# Autodesk Inventor assembly: Flyver
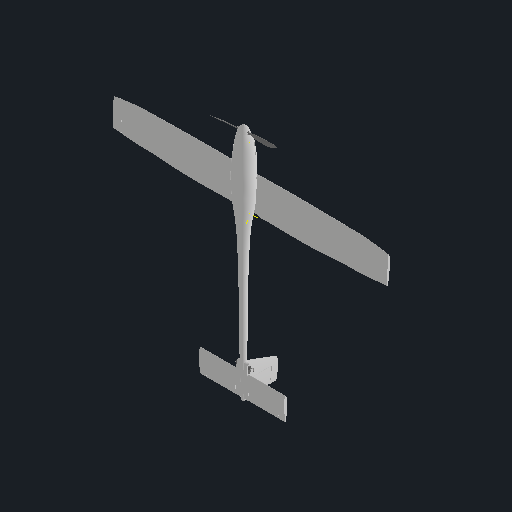
[picture p0: Inventor's stored thumbnail of the model, 512x512]
Saved by Autodesk Inventor 2026.2 (Build 302298000, 298)
## iProperties
Created: 2021-04-28
Part Number: Flyver
Document SubType Name: Assembly
Designer: armin
Author: armin
## Documents named in this file (19)
- C:\Users\Malthe Sennels\OneDrive - Aalborg Universitet\ESD 610 - General\Inventor\Cover_image\Flyver\Flyver.iam
- C:\Users\Malthe Sennels\OneDrive - Aalborg Universitet\ESD 610 - General\Inventor\Cover_image\Flyver\Body hollow.ipt
- C:\Users\Malthe Sennels\OneDrive - Aalborg Universitet\ESD 610 - General\Inventor\Cover_image\Flyver\Avionics.iam
- C:\Users\Malthe Sennels\OneDrive - Aalborg Universitet\ESD 610 - General\Inventor\Cover_image\Flyver\Wing.ipt
- C:\Users\Malthe Sennels\OneDrive - Aalborg Universitet\ESD 610 - General\Inventor\Cover_image\Flyver\Tunnel.ipt
- C:\Users\Malthe Sennels\OneDrive - Aalborg Universitet\ESD 610 - General\Inventor\Cover_image\Flyver\Servo.ipt
- C:\Users\Malthe Sennels\OneDrive - Aalborg Universitet\ESD 610 - General\Inventor\Cover_image\Flyver\Rudder.ipt
- C:\Users\Malthe Sennels\OneDrive - Aalborg Universitet\ESD 610 - General\Inventor\Cover_image\Flyver\Rudder_MIR.ipt
- C:\Users\Malthe Sennels\OneDrive - Aalborg Universitet\ESD 610 - General\Inventor\Cover_image\Flyver\Servo arm.ipt
- C:\Users\Malthe Sennels\OneDrive - Aalborg Universitet\ESD 610 - General\Inventor\Cover_image\Flyver\Styrepind.ipt
- C:\Users\Malthe Sennels\OneDrive - Aalborg Universitet\ESD 610 - General\Inventor\Cover_image\Flyver\BLDC.ipt
- C:\Users\Malthe Sennels\OneDrive - Aalborg Universitet\ESD 610 - General\Inventor\Cover_image\Flyver\Propeller.iam
- C:\Users\Malthe Sennels\OneDrive - Aalborg Universitet\ESD 610 - General\Inventor\Cover_image\Flyver\Servo_MIR.ipt
- C:\Users\Malthe Sennels\OneDrive - Aalborg Universitet\ESD 610 - General\Inventor\Cover_image\Flyver\Servo arm_MIR.ipt
- C:\Users\Malthe Sennels\OneDrive - Aalborg Universitet\ESD 610 - General\Inventor\Cover_image\Flyver\Styrepind_MIR.ipt
- C:\Users\Malthe Sennels\OneDrive - Aalborg Universitet\ESD 610 - General\Inventor\Cover_image\Flyver\Tail.ipt
- C:\Users\Malthe Sennels\OneDrive - Aalborg Universitet\ESD 610 - General\Inventor\Cover_image\Flyver\Aileron.ipt
- C:\Users\Malthe Sennels\OneDrive - Aalborg Universitet\ESD 610 - General\Inventor\Cover_image\Flyver\Wing_MIR1.ipt
- C:\Users\Malthe Sennels\OneDrive - Aalborg Universitet\ESD 610 - General\Inventor\Cover_image\Flyver\Aileron_MIR.ipt
## Components (19 placed, 18 different names)
1. Body hollow:1 — Mate:1, Mate:2, Mate:14, Mate:16, Mate:17, Mate:18, Mate:19, Mate:20, Flush:2, Flush:4, Flush:5, Mate:31, Mate:37, Mate:38, Flush:7, Mate:41, Mate:42, Mate:51
2. Avionics:1 [sub-assembly] — Mate:1, Mate:2, Mate:3, Mate:4, Flush:1, Mate:8, Mate:48, Mate:49, Mate:50, Mate:51
3. Wing:1 — Mate:3, Mate:4, Mate:8, Mate:44, Mate:45
4. Tunnel:1
5. Servo:1 — Mate:19, Mate:20, Flush:2, Mate:21, Mate:22
6. Rudder:1 — Mate:14, Mate:16, Mate:24
7. Rudder_MIR:1 — Mate:17, Mate:18, Mate:39
8. Servo arm:1 — Mate:21, Mate:22, Mate:23, Flush:3
9. Styrepind:1 — Mate:23, Mate:24, Flush:3
10. BLDC:1 — Mate:26, Mate:27, Mate:31, Mate:32, Mate:33, Mate:41
11. Propeller:1 [sub-assembly] — Mate:32, Mate:33
12. Servo_MIR:1 — Mate:34, Mate:35, Mate:37, Mate:38, Flush:7
13. Servo arm_MIR:1 — Mate:34, Mate:35, Flush:6, Mate:36
14. Styrepind_MIR:1 — Flush:6, Mate:36, Mate:39
15. Tail:1 — Mate:42
16. Aileron:1 — Mate:44, Mate:45
17. Wing_MIR1:1 — Mate:46, Mate:47, Mate:48, Mate:49, Mate:50
18. Aileron_MIR:1 — Mate:46, Mate:47
19. Tunnel:2
## Relationships (43: Mate 36, Flush 7)
- Mate:1: Body hollow:1 ↔ Avionics:1
- Mate:2: Body hollow:1 ↔ Avionics:1
- Mate:3: Avionics:1 ↔ Wing:1
- Mate:4: Avionics:1 ↔ Wing:1
- Flush:1 (-5 mm): Avionics:1
- Mate:8: Avionics:1 ↔ Wing:1
- Mate:14: Body hollow:1 ↔ Rudder:1
- Mate:16 (1 mm): Body hollow:1 ↔ Rudder:1
- Mate:17: Body hollow:1 ↔ Rudder_MIR:1
- Mate:18 (1 mm): Body hollow:1 ↔ Rudder_MIR:1
- Mate:19: Body hollow:1 ↔ Servo:1
- Mate:20: Body hollow:1 ↔ Servo:1
- Flush:2: Body hollow:1 ↔ Servo:1
- Mate:21: Servo:1 ↔ Servo arm:1
- Mate:22: Servo:1 ↔ Servo arm:1
- Mate:23: Servo arm:1 ↔ Styrepind:1
- Mate:24: Rudder:1 ↔ Styrepind:1
- Flush:3: Servo arm:1 ↔ Styrepind:1
- Flush:4 (-25 mm): Body hollow:1
- Mate:26: BLDC:1
- Mate:27: BLDC:1
- Flush:5 (-182 mm): Body hollow:1
- Mate:31: Body hollow:1 ↔ BLDC:1
- Mate:32: BLDC:1 ↔ Propeller:1
- Mate:33: BLDC:1 ↔ Propeller:1
- Mate:34: Servo_MIR:1 ↔ Servo arm_MIR:1
- Mate:35: Servo_MIR:1 ↔ Servo arm_MIR:1
- Flush:6: Servo arm_MIR:1 ↔ Styrepind_MIR:1
- Mate:36: Servo arm_MIR:1 ↔ Styrepind_MIR:1
- Mate:37: Body hollow:1 ↔ Servo_MIR:1
- Mate:38: Body hollow:1 ↔ Servo_MIR:1
- Flush:7: Body hollow:1 ↔ Servo_MIR:1
- Mate:39: Rudder_MIR:1 ↔ Styrepind_MIR:1
- Mate:41: Body hollow:1 ↔ BLDC:1
- Mate:42: Body hollow:1 ↔ Tail:1
- Mate:44: Wing:1 ↔ Aileron:1
- Mate:45 (1 mm): Wing:1 ↔ Aileron:1
- Mate:46 (1 mm): Wing_MIR1:1 ↔ Aileron_MIR:1
- Mate:47: Wing_MIR1:1 ↔ Aileron_MIR:1
- Mate:48: Avionics:1 ↔ Wing_MIR1:1
- Mate:49: Avionics:1 ↔ Wing_MIR1:1
- Mate:50: Avionics:1 ↔ Wing_MIR1:1
- Mate:51: Body hollow:1 ↔ Avionics:1
